# Autodesk Inventor assembly: 2AM-17-A-0200 - slider motor and gearbox
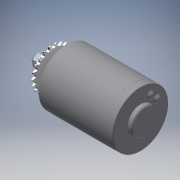
[picture p0: Inventor's stored thumbnail of the model, 180x180]
Saved by Autodesk Inventor 2017 (Build 210142000, 142)
## iProperties
Created: 2017-12-28
Part Number: 2AM-17-A-0200 - slider motor and gearbox
Document SubType Name: Assembly
Designer: Micah
Author: Micah
## Documents named in this file (5)
- C:\Users\Micah\Desktop\inventor\CADathon-2017\2AM-17-A-0200 - Smokestack Elevator\2AM-17-A-0200 - slider motor and gearbox.iam
- C:\Users\Micah\Desktop\inventor\COTS\Motors\Mini CIM Motor\217-3371-STEP.ipt
- C:\Users\Micah\Desktop\inventor\CADathon-2017\2AM-17-A-0200 - Smokestack Elevator\COTS\217-2761-STEP.ipt
- C:\Users\Micah\Desktop\inventor\CADathon-2017\2AM-17-A-0200 - Smokestack Elevator\COTS\217-3255-STEP.ipt
- C:\Users\Micah\Desktop\inventor\CADathon-2017\2AM-17-A-0200 - Smokestack Elevator\COTS\_22t_Aluminum_Hub_Sprocket_25_Chain_1_2_Hex_Bore_217-2640.ipt
## Components (4 placed, 4 different names)
1. 217-3371-STEP:1 — Mate:1, Insert:1, Rotational:1
2. 217-2761-STEP:2 — Mate:1
3. 217-3255-STEP:1 — Insert:1
4. _22t_Aluminum_Hub_Sprocket_25_Chain_1_2_Hex_Bore_217-2640:1 — Rotational:1
## Relationships (3: Mate 1, Insert 1, RevoluteJoint 1)
- Mate:1: 217-3371-STEP:1 ↔ 217-2761-STEP:2
- Insert:1 (-28.575 mm): 217-3371-STEP:1 ↔ 217-3255-STEP:1
- Rotational:1 [RevoluteJoint] (-12.7 mm): 217-3371-STEP:1 ↔ _22t_Aluminum_Hub_Sprocket_25_Chain_1_2_Hex_Bore_217-2640:1
